# Autodesk Inventor assembly: Form
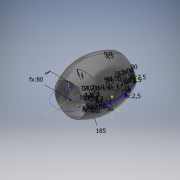
[picture p0: Inventor's stored thumbnail of the model, 180x180]
Saved by Autodesk Inventor 2018.3 (Build 223284000, 284)
## iProperties
Created: 2018-07-24
Part Number: Form
Material: Generisch
Document SubType Name: Assembly
Designer: JochenAlt
Author: JochenAlt
## Documents named in this file (6)
- D:\Projects\FlowerPot\CAD\Form.iam
- D:\Projects\FlowerPot\CAD\Form.ipt
- D:\Projects\FlowerPot\CAD\Spindle\Spindle.ipt
- D:\Projects\FlowerPot\CAD\Spindle\W 61700 X-2RS1.iam
- D:\Projects\FlowerPot\CAD\Spindle\SpindleWithGear.ipt
- D:\Projects\FlowerPot\CAD\SpindleMotor.iam
## Components (11 placed, 4 different names)
1. Form:1 — Passend:13, Passend:14, Passend:15, Passend:16, Passend:17, Passend:18, Passend:21, Passend:22
2. Spindle:1 — Passend:1, Passend:4, Passend:11, Passend:12
3. Spindle:2 — Passend:2, Passend:3, Passend:9, Passend:16, Passend:20
4. Spindle:3 — Passend:5, Passend:6, Passend:7, Passend:17, Passend:19
5. W 61700 X-2RS1:1 [sub-assembly] — Passend:1, Passend:12, Passend:13, Passend:18
6. W 61700 X-2RS1:2 [sub-assembly] — Passend:2, Passend:9, Passend:15
7. W 61700 X-2RS1:3 [sub-assembly] — Passend:6, Passend:19
8. W 61700 X-2RS1:4 [sub-assembly] — Passend:5, Passend:7, Passend:14
9. W 61700 X-2RS1:5 [sub-assembly] — Passend:3, Passend:20
10. W 61700 X-2RS1:6 [sub-assembly] — Passend:4, Passend:11
11. SpindleMotor:1 [sub-assembly] — Passend:21, Passend:22
## Relationships (20: Mate 20)
- Passend:1 [Mate]: Spindle:1 ↔ W 61700 X-2RS1:1
- Passend:2 [Mate]: Spindle:2 ↔ W 61700 X-2RS1:2
- Passend:3 [Mate]: Spindle:2 ↔ W 61700 X-2RS1:5
- Passend:4 [Mate]: Spindle:1 ↔ W 61700 X-2RS1:6
- Passend:5 [Mate]: Spindle:3 ↔ W 61700 X-2RS1:4
- Passend:6 [Mate]: Spindle:3 ↔ W 61700 X-2RS1:3
- Passend:7 [Mate]: Spindle:3 ↔ W 61700 X-2RS1:4
- Passend:9 [Mate]: Spindle:2 ↔ W 61700 X-2RS1:2
- Passend:11 [Mate]: Spindle:1 ↔ W 61700 X-2RS1:6
- Passend:12 [Mate]: Spindle:1 ↔ W 61700 X-2RS1:1
- Passend:13 [Mate]: Form:1 ↔ W 61700 X-2RS1:1
- Passend:14 [Mate]: Form:1 ↔ W 61700 X-2RS1:4
- Passend:15 [Mate]: Form:1 ↔ W 61700 X-2RS1:2
- Passend:16 [Mate]: Form:1 ↔ Spindle:2
- Passend:17 [Mate]: Form:1 ↔ Spindle:3
- Passend:18 [Mate]: Form:1 ↔ W 61700 X-2RS1:1
- Passend:19 [Mate]: Spindle:3 ↔ W 61700 X-2RS1:3
- Passend:20 [Mate]: Spindle:2 ↔ W 61700 X-2RS1:5
- Passend:21 [Mate]: Form:1 ↔ SpindleMotor:1
- Passend:22 [Mate]: Form:1 ↔ SpindleMotor:1
